# Autodesk Inventor assembly: SUPPORT_MIR
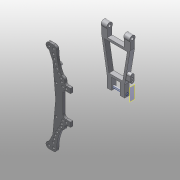
[picture p0: Inventor's stored thumbnail of the model, 180x180]
Saved by Autodesk Inventor 2015 (Build 190159000, 159)
## iProperties
Created: 2015-04-18
Part Number: SUPPORT_MIR
Document SubType Name: Assembly
Designer: Station9
Author: Station9
## Documents named in this file (5)
- D:\Project Archive\AD\AD-6(94.01.29)WSC2011\SUPPORT_MIR.iam
- D:\Project Archive\AD\AD-6(94.01.29)WSC2011\500-006_MIR.ipt
- D:\Project Archive\AD\AD-6(94.01.29)WSC2011\307-320_MIR.ipt
- D:\Project Archive\AD\AD-6(94.01.29)WSC2011\500-111_MIR.ipt
- D:\Project Archive\AD\AD-6(94.01.29)WSC2011\500-120_MIR.ipt
## Components (4 placed, 4 different names)
1. 500-006_MIR:1 — Flush:1, Mate:1
2. 307-320_MIR:1 — Flush:1, Mate:1
3. 500-111_MIR:1
4. 500-120_MIR:1
## Relationships (2: Flush 1, Mate 1)
- Flush:1: 500-006_MIR:1 ↔ 307-320_MIR:1
- Mate:1: 500-006_MIR:1 ↔ 307-320_MIR:1
